# Autodesk Inventor assembly: 276-2216
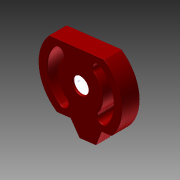
[picture p0: Inventor's stored thumbnail of the model, 180x180]
Saved by Autodesk Inventor 2013 (Build 170138000, 138)
## iProperties
Category: Sensors
Company: Autodesk Inc.
Created: 2012-04-09
Part Number: 276-2216
Document SubType Name: Assembly
Designer: Autodesk Inc.
Catalog Web Link: http://www.vexrobotics.com/276-2216.html
Vendor: VEX
Mass: 18.1437 g
Surface Area: 75.8524 cm^2
Volume: 3.81724 cm^3
Author: Autodesk Inc.
## Documents named in this file (4)
- C:\Data Folder\VEX 2012\VEX KOP Uploads\2013\Metric\Sensors\Potentiometer.iam
- C:\Data Folder\VEX 2012\VEX KOP Uploads\2013\Metric\Sensors\Components\Potentiometer Sensor.ipt
- C:\Data Folder\VEX 2012\VEX KOP Uploads\2013\Metric\Sensors\Components\Potentiometer Back.ipt
- C:\Data Folder\VEX 2012\VEX KOP Uploads\2013\Metric\Sensors\Components\Potentiometer Front.ipt
## Components (3 placed, 3 different names)
1. Potentiometer Sensor:1 — Mate:1, Mate:2, Mate:3
2. Potentiometer Back:1 — Mate:3, Mate:4, Flush:1
3. Potentiometer Front:1 — Mate:1, Mate:2, Mate:4, Flush:1
## Relationships (5: Mate 4, Flush 1)
- Mate:1: Potentiometer Sensor:1 ↔ Potentiometer Front:1
- Mate:2: Potentiometer Sensor:1 ↔ Potentiometer Front:1
- Mate:3: Potentiometer Sensor:1 ↔ Potentiometer Back:1
- Mate:4: Potentiometer Back:1 ↔ Potentiometer Front:1
- Flush:1: Potentiometer Back:1 ↔ Potentiometer Front:1
